# Autodesk Inventor assembly: Robot
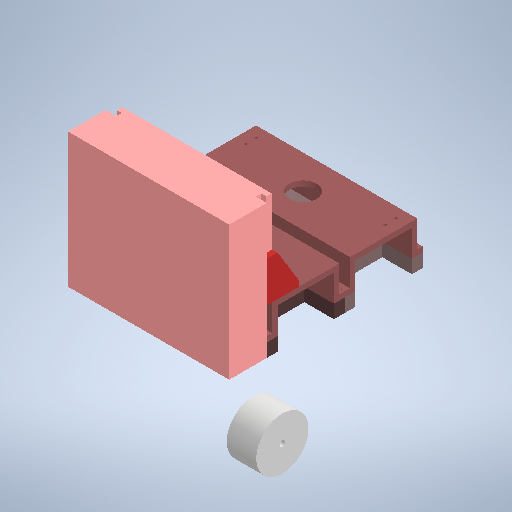
[picture p0: Inventor's stored thumbnail of the model, 512x512]
Saved by Autodesk Inventor 2025.3 (Build 293356000, 356)
## iProperties
Created: 2025-04-27
Part Number: Robot
Document SubType Name: Assembly
Designer: SEON
Author: SEON
## Documents named in this file (6)
- C:\Users\SEON\Documents\Inventor\LastCapstone\Robot.iam
- C:\Users\SEON\Documents\Inventor\LastCapstone\DummyModule.ipt
- C:\Users\SEON\Documents\Inventor\LastCapstone\RobotBase.ipt
- C:\Users\SEON\Documents\Inventor\LastCapstone\ModuleConnector.ipt
- C:\Users\SEON\Documents\Inventor\LastCapstone\DummyWheel.ipt
- C:\Users\SEON\Documents\Inventor\LastCapstone\WheelCorver.ipt
## Components (9 placed, 5 different names)
1. RobotBase:1 — 메이트:1, 메이트:4, 메이트:5, 메이트:6, 플러쉬:3, 메이트:9, 플러쉬:4, 메이트:11, 메이트:12, 플러쉬:5, 플러쉬:6, 메이트:13, 플러쉬:8
2. DummyModule:1 — 메이트:6, 메이트:8, 메이트:18, 메이트:19
3. ModuleConnector:1 — 플러쉬:3, 메이트:8, 메이트:10, 메이트:16, 메이트:18, 메이트:19
4. DummyWheel:1 — 각도:1
5. WheelCorver:1 — 메이트:9, 메이트:10, 플러쉬:4, 메이트:16, 플러쉬:10, 플러쉬:11, 메이트:17
6. WheelCorver:2 — 메이트:11, 플러쉬:11, 메이트:17
7. RobotBase:2 — 메이트:13, 메이트:15, 플러쉬:7, 플러쉬:8, 플러쉬:10
8. RobotBase:3 — 메이트:14, 메이트:15, 플러쉬:7, 플러쉬:9
9. RobotBase:4 — 메이트:12, 플러쉬:5, 플러쉬:6, 메이트:14, 플러쉬:9
## Relationships (26: Mate 16, Flush 9, Angle 1)
- 메이트:1 [Mate]: RobotBase:1
- 메이트:4 [Mate]: RobotBase:1
- 메이트:5 [Mate]: RobotBase:1
- 메이트:6 [Mate]: RobotBase:1 ↔ DummyModule:1
- 플러쉬:3 [Flush]: RobotBase:1 ↔ ModuleConnector:1
- 메이트:8 [Mate]: DummyModule:1 ↔ ModuleConnector:1
- 각도:1 [Angle] (0 deg): DummyWheel:1
- 메이트:9 [Mate]: RobotBase:1 ↔ WheelCorver:1
- 메이트:10 [Mate]: ModuleConnector:1 ↔ WheelCorver:1
- 플러쉬:4 [Flush]: RobotBase:1 ↔ WheelCorver:1
- 메이트:11 [Mate]: RobotBase:1 ↔ WheelCorver:2
- 메이트:12 [Mate]: RobotBase:1 ↔ RobotBase:4
- 플러쉬:5 [Flush]: RobotBase:1 ↔ RobotBase:4
- 플러쉬:6 [Flush]: RobotBase:1 ↔ RobotBase:4
- 메이트:13 [Mate]: RobotBase:1 ↔ RobotBase:2
- 메이트:14 [Mate]: RobotBase:3 ↔ RobotBase:4
- 메이트:15 [Mate]: RobotBase:2 ↔ RobotBase:3
- 플러쉬:7 [Flush]: RobotBase:2 ↔ RobotBase:3
- 플러쉬:8 [Flush]: RobotBase:1 ↔ RobotBase:2
- 플러쉬:9 [Flush]: RobotBase:3 ↔ RobotBase:4
- 메이트:16 [Mate]: ModuleConnector:1 ↔ WheelCorver:1
- 플러쉬:10 [Flush]: WheelCorver:1 ↔ RobotBase:2
- 플러쉬:11 [Flush]: WheelCorver:1 ↔ WheelCorver:2
- 메이트:17 [Mate]: WheelCorver:1 ↔ WheelCorver:2
- 메이트:18 [Mate]: DummyModule:1 ↔ ModuleConnector:1
- 메이트:19 [Mate]: DummyModule:1 ↔ ModuleConnector:1
